# Autodesk Inventor assembly: 08-00-00-000_TurnGTAssembly_Auxilary
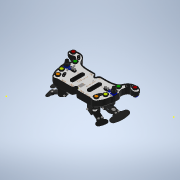
[picture p0: Inventor's stored thumbnail of the model, 180x180]
Saved by Autodesk Inventor 2020 (Build 240168000, 168)
## iProperties
Created: 2021-07-25
Part Number: 08-00-00-000_TurnGTAssembly_Auxilary
Document SubType Name: Assembly
Designer: Eric
Mass: 544.726 g
Surface Area: 2233.35 cm^2
Volume: 211.21 cm^3
Density: 2.57907 g/cm^3
Author: Eric
## Documents named in this file (13)
- C:\Users\Eric\Documents\repos\DIY_CAD_WheelButtonPlate\CAD\Inventor\08-00-00-000_TurnGTAssembly_Auxilary.iam
- C:\Users\Eric\Documents\repos\DIY_CAD_WheelButtonPlate\CAD\Inventor\08-03-00-000_TurnGTElectronics.iam
- C:\Users\Eric\Documents\repos\DIY_CAD_WheelButtonPlate\CAD\Inventor\08-02-01-002_SteeringWheelSpacer.ipt
- C:\Users\Eric\Documents\repos\DIY_CAD_WheelButtonPlate\CAD\Inventor\08-02-01-004_backCover.ipt
- C:\Users\Eric\Documents\repos\DIY_CAD_WheelButtonPlate\CAD\Inventor\08-04-00-000_clutchPaddleAssembly.iam
- C:\Users\Eric\Documents\repos\DIY_CAD_WheelButtonPlate\CAD\Inventor\08-04-01-006_clutchPaddle.ipt
- C:\Users\Eric\Documents\repos\DIY_CAD_WheelButtonPlate\CAD\Inventor\08-02-01-010_buttonSide.ipt
- C:\Users\Eric\Documents\repos\DIY_CAD_WheelButtonPlate\CAD\Inventor\08-02-01-011_funkyKnob.ipt
- C:\Users\Eric\Documents\repos\DIY_CAD_WheelButtonPlate\CAD\Inventor\08-02-01-012_SteeringWheelSpacerLeft.ipt
- C:\Users\Eric\Documents\repos\DIY_CAD_WheelButtonPlate\CAD\Inventor\04-00-02-006_Apem_blue.ipt
- C:\Users\Eric\Documents\repos\DIY_CAD_WheelButtonPlate\CAD\Inventor\08-02-01-014_funkySide.ipt
- C:\Users\Eric\Documents\repos\DIY_CAD_WheelButtonPlate\CAD\Inventor\08-05-00-000_shifter_assembly.iam
- C:\Users\Eric\Documents\repos\DIY_CAD_WheelButtonPlate\CAD\Inventor\08-06-00-000_GX12-6P_assembly.iam
## Components (24 placed, 12 different names)
1. 08-03-00-000_TurnGTElectronics:1 [sub-assembly] — Passend:55, Passend:56, Passend:57, Passend:58, Passend:59, Passend:60, Passend:106, Passend:107, Passend:108, Passend:109, Passend:110, Passend:111, Passend:112, Passend:113
2. 08-02-01-002_SteeringWheelSpacer:1 — Passend:15, Passend:34, Passend:35
3. 08-02-01-004_backCover:1 — Passend:15, Passend:66, Passend:69, Passend:82, Passend:85, Passend:86, Passend:88, Passend:89, Passend:91, Passend:92, Passend:100, Passend:101, Passend:102, Passend:103, Passend:104, Passend:105
4. 08-04-00-000_clutchPaddleAssembly:1 [sub-assembly] — Passend:64, Passend:65
5. 08-04-00-000_clutchPaddleAssembly:2 [sub-assembly] — Passend:34, Passend:35, Passend:37, Passend:38, Passend:39
6. 08-04-01-006_clutchPaddle:1 — Passend:37, Passend:38, Passend:39
7. 08-02-01-010_buttonSide:1 — Passend:106, Fluchtend:10, Fluchtend:11
8. 08-02-01-011_funkyKnob:1 — Passend:55, Passend:56, Passend:57
9. 08-02-01-011_funkyKnob:2 — Passend:58, Passend:59, Passend:60
10. 08-02-01-012_SteeringWheelSpacerLeft:1 — Passend:64, Passend:65, Passend:69
11. 08-06-00-000_GX12-6P_assembly:1 [sub-assembly] — Passend:66, Passend:82
12. 08-02-01-010_buttonSide:3 — Fluchtend:9, Passend:107, Fluchtend:11
13. 08-02-01-010_buttonSide:4 — Fluchtend:7, Fluchtend:8, Passend:112
14. 08-02-01-010_buttonSide:5 — Fluchtend:6, Fluchtend:7, Passend:110
15. 08-02-01-010_buttonSide:6 — Fluchtend:8, Fluchtend:9, Passend:113
16. 08-02-01-010_buttonSide:7 — Fluchtend:3, Passend:111
17. 08-02-01-010_buttonSide:8 — Fluchtend:3, Passend:108, Fluchtend:12
18. 08-02-01-010_buttonSide:10 — Fluchtend:6, Fluchtend:12, Passend:109
19. 04-00-02-006_Apem_blue:1 — Passend:85, Passend:86, Passend:91
20. 04-00-02-006_Apem_blue:2 — Passend:88, Passend:89, Passend:92
21. 08-02-01-014_funkySide:1
22. 08-02-01-014_funkySide:2 — Fluchtend:10
23. 08-05-00-000_shifter_assembly:1 [sub-assembly] — Passend:103, Passend:104, Passend:105
24. 08-05-00-000_shifter_assembly:2 [sub-assembly] — Passend:100, Passend:101, Passend:102
## Relationships (45: Mate 37, Flush 8)
- Passend:15 [Mate]: 08-02-01-002_SteeringWheelSpacer:1 ↔ 08-02-01-004_backCover:1
- Passend:34 [Mate]: 08-02-01-002_SteeringWheelSpacer:1 ↔ 08-04-00-000_clutchPaddleAssembly:2
- Passend:35 [Mate]: 08-02-01-002_SteeringWheelSpacer:1 ↔ 08-04-00-000_clutchPaddleAssembly:2
- Passend:37 [Mate]: 08-04-00-000_clutchPaddleAssembly:2 ↔ 08-04-01-006_clutchPaddle:1
- Passend:38 [Mate]: 08-04-00-000_clutchPaddleAssembly:2 ↔ 08-04-01-006_clutchPaddle:1
- Passend:39 [Mate]: 08-04-00-000_clutchPaddleAssembly:2 ↔ 08-04-01-006_clutchPaddle:1
- Passend:55 [Mate]: 08-03-00-000_TurnGTElectronics:1 ↔ 08-02-01-011_funkyKnob:1
- Passend:56 [Mate]: 08-03-00-000_TurnGTElectronics:1 ↔ 08-02-01-011_funkyKnob:1
- Passend:57 [Mate]: 08-03-00-000_TurnGTElectronics:1 ↔ 08-02-01-011_funkyKnob:1
- Passend:58 [Mate]: 08-03-00-000_TurnGTElectronics:1 ↔ 08-02-01-011_funkyKnob:2
- Passend:59 [Mate]: 08-03-00-000_TurnGTElectronics:1 ↔ 08-02-01-011_funkyKnob:2
- Passend:60 [Mate]: 08-03-00-000_TurnGTElectronics:1 ↔ 08-02-01-011_funkyKnob:2
- Passend:64 [Mate]: 08-04-00-000_clutchPaddleAssembly:1 ↔ 08-02-01-012_SteeringWheelSpacerLeft:1
- Passend:65 [Mate]: 08-04-00-000_clutchPaddleAssembly:1 ↔ 08-02-01-012_SteeringWheelSpacerLeft:1
- Passend:66 [Mate]: 08-02-01-004_backCover:1 ↔ 08-06-00-000_GX12-6P_assembly:1
- Passend:69 [Mate]: 08-02-01-004_backCover:1 ↔ 08-02-01-012_SteeringWheelSpacerLeft:1
- Fluchtend:3 [Flush]: 08-02-01-010_buttonSide:7 ↔ 08-02-01-010_buttonSide:8
- Fluchtend:6 [Flush]: 08-02-01-010_buttonSide:5 ↔ 08-02-01-010_buttonSide:10
- Fluchtend:7 [Flush]: 08-02-01-010_buttonSide:4 ↔ 08-02-01-010_buttonSide:5
- Fluchtend:8 [Flush]: 08-02-01-010_buttonSide:4 ↔ 08-02-01-010_buttonSide:6
- Fluchtend:9 [Flush]: 08-02-01-010_buttonSide:3 ↔ 08-02-01-010_buttonSide:6
- Passend:82 [Mate] (28.5 mm): 08-02-01-004_backCover:1 ↔ 08-06-00-000_GX12-6P_assembly:1
- Passend:85 [Mate]: 08-02-01-004_backCover:1 ↔ 04-00-02-006_Apem_blue:1
- Passend:86 [Mate]: 08-02-01-004_backCover:1 ↔ 04-00-02-006_Apem_blue:1
- Passend:88 [Mate]: 08-02-01-004_backCover:1 ↔ 04-00-02-006_Apem_blue:2
- Passend:89 [Mate]: 08-02-01-004_backCover:1 ↔ 04-00-02-006_Apem_blue:2
- Passend:91 [Mate]: 08-02-01-004_backCover:1 ↔ 04-00-02-006_Apem_blue:1
- Passend:92 [Mate]: 08-02-01-004_backCover:1 ↔ 04-00-02-006_Apem_blue:2
- Passend:100 [Mate]: 08-02-01-004_backCover:1 ↔ 08-05-00-000_shifter_assembly:2
- Passend:101 [Mate]: 08-02-01-004_backCover:1 ↔ 08-05-00-000_shifter_assembly:2
- Passend:102 [Mate]: 08-02-01-004_backCover:1 ↔ 08-05-00-000_shifter_assembly:2
- Passend:103 [Mate]: 08-02-01-004_backCover:1 ↔ 08-05-00-000_shifter_assembly:1
- Passend:104 [Mate]: 08-02-01-004_backCover:1 ↔ 08-05-00-000_shifter_assembly:1
- Passend:105 [Mate]: 08-02-01-004_backCover:1 ↔ 08-05-00-000_shifter_assembly:1
- Passend:106 [Mate]: 08-03-00-000_TurnGTElectronics:1 ↔ 08-02-01-010_buttonSide:1
- Fluchtend:10 [Flush]: 08-02-01-010_buttonSide:1 ↔ 08-02-01-014_funkySide:2
- Passend:107 [Mate]: 08-03-00-000_TurnGTElectronics:1 ↔ 08-02-01-010_buttonSide:3
- Fluchtend:11 [Flush]: 08-02-01-010_buttonSide:1 ↔ 08-02-01-010_buttonSide:3
- Passend:108 [Mate]: 08-03-00-000_TurnGTElectronics:1 ↔ 08-02-01-010_buttonSide:8
- Fluchtend:12 [Flush]: 08-02-01-010_buttonSide:8 ↔ 08-02-01-010_buttonSide:10
- Passend:109 [Mate]: 08-03-00-000_TurnGTElectronics:1 ↔ 08-02-01-010_buttonSide:10
- Passend:110 [Mate]: 08-03-00-000_TurnGTElectronics:1 ↔ 08-02-01-010_buttonSide:5
- Passend:111 [Mate]: 08-03-00-000_TurnGTElectronics:1 ↔ 08-02-01-010_buttonSide:7
- Passend:112 [Mate]: 08-03-00-000_TurnGTElectronics:1 ↔ 08-02-01-010_buttonSide:4
- Passend:113 [Mate]: 08-03-00-000_TurnGTElectronics:1 ↔ 08-02-01-010_buttonSide:6
